# Autodesk Inventor assembly: Catapult
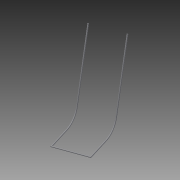
[picture p0: Inventor's stored thumbnail of the model, 180x180]
Saved by Autodesk Inventor 2013 (Build 170138000, 138)
## iProperties
Created: 2014-01-21
Part Number: Catapult
Document SubType Name: Assembly
Designer: robotics
Author: robotics
## Documents named in this file (3)
- C:\team3566-2014\CAD\Catapult.iam
- C:\team3566-2014\CAD\Catapult Arm 1.ipt
- C:\team3566-2014\CAD\Catapult End.ipt
## Components (3 placed, 2 different names)
1. Catapult Arm 1:1 — Insert:2, Angle:1, Angle:3, Angle:5, Insert:4
2. Catapult Arm 1:2 — Insert:1, Angle:2, Angle:4, Angle:5, Insert:3
3. Catapult End:1 — Insert:1, Insert:2, Angle:1, Angle:2, Angle:3, Angle:4, Insert:3, Insert:4
## Relationships (9: Angle 5, Insert 4)
- Insert:1: Catapult Arm 1:2 ↔ Catapult End:1
- Insert:2: Catapult Arm 1:1 ↔ Catapult End:1
- Angle:1 (0 deg): Catapult Arm 1:1 ↔ Catapult End:1
- Angle:2 (90 deg): Catapult Arm 1:2 ↔ Catapult End:1
- Angle:3 (270 deg): Catapult Arm 1:1 ↔ Catapult End:1
- Angle:4 (90 deg): Catapult Arm 1:2 ↔ Catapult End:1
- Angle:5 (0 deg): Catapult Arm 1:1 ↔ Catapult Arm 1:2
- Insert:3: Catapult Arm 1:2 ↔ Catapult End:1
- Insert:4: Catapult Arm 1:1 ↔ Catapult End:1
